# Autodesk Inventor assembly: Zespół1
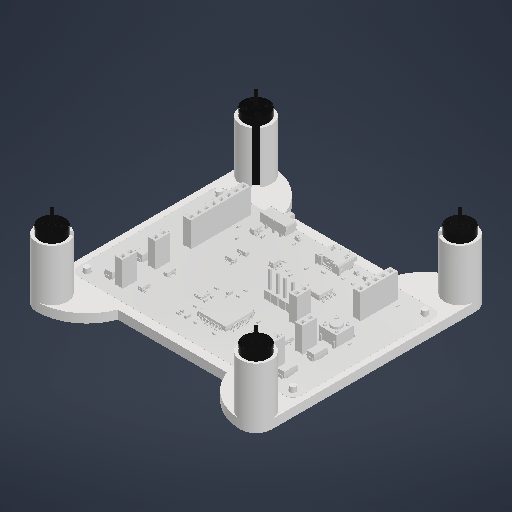
[picture p0: Inventor's stored thumbnail of the model, 512x512]
Saved by Autodesk Inventor 2026.2 (Build 302298000, 298)
## iProperties
Created: 2026-01-10
Part Number: Zespół1
Document SubType Name: Assembly
Designer: DeathLock
Author: DeathLock
## Documents named in this file (4)
- C:\Users\mjank\Documents\GitHub\STM32-Drone\Drone_3D\Zespół1.iam
- C:\Users\mjank\Documents\GitHub\STM32-Drone\Drone_3D\8520 Coreless Brshed motor.ipt
- C:\Users\mjank\Documents\GitHub\STM32-Drone\Drone_3D\Drone.ipt
- C:\Users\mjank\Documents\GitHub\STM32-Drone\Drone_3D\Drone_PCB.ipt
## Components (6 placed, 3 different names)
1. Drone:1 — Sztywne:1, Sztywne:2, Sztywne:3, Sztywne:4, Sztywne:5, Sztywne:6, Sztywne:7, Sztywne:8, Sztywne:9, Sztywne:10
2. Drone_PCB:1 — Sztywne:1, Sztywne:6
3. 8520 Coreless Brshed motor:1 — Sztywne:3, Sztywne:9
4. 8520 Coreless Brshed motor:2 — Sztywne:4, Sztywne:7
5. 8520 Coreless Brshed motor:3 — Sztywne:5, Sztywne:10
6. 8520 Coreless Brshed motor:4 — Sztywne:2, Sztywne:8
## Relationships (10: WeldJoint 10)
- Sztywne:1 [WeldJoint]: Drone:1 ↔ Drone_PCB:1
- Sztywne:2 [WeldJoint]: Drone:1 ↔ 8520 Coreless Brshed motor:4
- Sztywne:3 [WeldJoint]: Drone:1 ↔ 8520 Coreless Brshed motor:1
- Sztywne:4 [WeldJoint]: Drone:1 ↔ 8520 Coreless Brshed motor:2
- Sztywne:5 [WeldJoint]: Drone:1 ↔ 8520 Coreless Brshed motor:3
- Sztywne:6 [WeldJoint]: Drone:1 ↔ Drone_PCB:1
- Sztywne:7 [WeldJoint]: Drone:1 ↔ 8520 Coreless Brshed motor:2
- Sztywne:8 [WeldJoint]: Drone:1 ↔ 8520 Coreless Brshed motor:4
- Sztywne:9 [WeldJoint]: Drone:1 ↔ 8520 Coreless Brshed motor:1
- Sztywne:10 [WeldJoint]: Drone:1 ↔ 8520 Coreless Brshed motor:3
